# Autodesk Inventor assembly: MG_996R
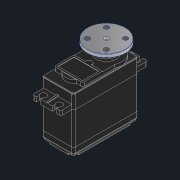
[picture p0: Inventor's stored thumbnail of the model, 180x180]
Saved by Autodesk Inventor 2022 (Build 260153000, 153)
## iProperties
Created: 2016-09-26
Part Number: MG_996R
Document SubType Name: Assembly
Designer: Julian
Mass: 36.0153 g
Surface Area: 118.599 cm^2
Volume: 31.6169 cm^3
Density: 1.13912 g/cm^3
Author: Julian
## Documents named in this file (6)
- C:\Users\yuta0\Documents\GitHub\catchrobo_hardware\assy-robot\MG_996R.iam
- C:\Users\yuta0\Documents\GitHub\catchrobo_hardware\assy-robot\servo_Base.ipt
- C:\Users\yuta0\Documents\GitHub\catchrobo_hardware\assy-robot\Medio.ipt
- C:\Users\yuta0\Documents\GitHub\catchrobo_hardware\assy-robot\Top.ipt
- C:\Users\yuta0\Documents\GitHub\catchrobo_hardware\assy-robot\Eje.ipt
- C:\Users\yuta0\Documents\GitHub\catchrobo_hardware\assy-robot\horn.ipt
## Components (5 placed, 5 different names)
1. Top:1 — De rotación:1, メイト:3, メイト:4, メイト:5, メイト:10, メイト:11, フラッシュ:1, メイト:12, メイト:13
2. Medio:1 — メイト:3, メイト:4, メイト:5, メイト:6, メイト:7, メイト:8, 角度:2
3. servo_Base:1 — メイト:6, メイト:7, メイト:8
4. Eje:1 — De rotación:1
5. horn:1 — メイト:10, メイト:11, 角度:1
## Relationships (14: Mate 10, Angle 2, RevoluteJoint 1, Flush 1)
- De rotación:1 [RevoluteJoint]: Top:1 ↔ Eje:1
- メイト:3 [Mate]: Top:1 ↔ Medio:1
- メイト:4 [Mate]: Top:1 ↔ Medio:1
- メイト:5 [Mate]: Top:1 ↔ Medio:1
- メイト:6 [Mate]: Medio:1 ↔ servo_Base:1
- メイト:7 [Mate]: Medio:1 ↔ servo_Base:1
- メイト:8 [Mate]: Medio:1 ↔ servo_Base:1
- メイト:10 [Mate]: Top:1 ↔ horn:1
- メイト:11 [Mate]: Top:1 ↔ horn:1
- 角度:1 [Angle] (45 deg): horn:1
- 角度:2 [Angle] (0 deg): Medio:1
- フラッシュ:1 [Flush]: Top:1
- メイト:12 [Mate]: Top:1
- メイト:13 [Mate]: Top:1
